# Autodesk Inventor assembly: Gripper2
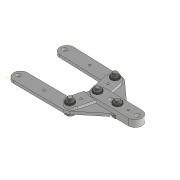
[picture p0: Inventor's stored thumbnail of the model, 180x180]
Saved by Autodesk Inventor 2021 (Build 250183000, 183)
## iProperties
Created: 2022-10-02
Part Number: Gripper2
Document SubType Name: Assembly
Designer: brian
Author: brian
## Documents named in this file (8)
- G:\Mi unidad\Universidad\Control\Robotica\Laboratorio\Proyecto\Gripper2.iam
- G:\Mi unidad\Universidad\Control\Robotica\Laboratorio\Proyecto\GripP1.ipt
- G:\Mi unidad\Universidad\Control\Robotica\Laboratorio\Proyecto\GripP3.ipt
- G:\Mi unidad\Universidad\Control\Robotica\Laboratorio\Proyecto\GripP4.ipt
- C:\Users\brian\OneDrive\Documents\Inventor\Content Center Files\R2021\en-US\ISO 8738(2)\ISO 8738 - 10(2).ipt
- C:\Users\brian\OneDrive\Documents\Inventor\Content Center Files\R2021\en-US\ISO 4017(1)\ISO 4017 - M10 x 20 - ISO.ipt
- C:\Users\brian\OneDrive\Documents\Inventor\Content Center Files\R2021\en-US\ISO 4017(1)\ISO 4017 - M10 x 25 - ISO.ipt
- C:\Users\brian\OneDrive\Documents\Inventor\Content Center Files\R2021\en-US\ISO 8675(2)\ISO 8675 - M8 x 1 - ISO.ipt
## Components (21 placed, 7 different names)
1. GripP1:1 — Rotational:5, Rotational:7, Insert:1, Insert:4
2. GripP3:1 — Rotational:3, Rotational:5, Rotational:6, Insert:10
3. GripP1:2 — Rotational:4, Rotational:7, Tangent:1, Insert:3
4. GripP3:2 — Rotational:3, Rotational:4, Insert:2, Insert:11
5. GripP4:2 — Rotational:6, Tangent:1, Insert:6
6. ISO 8738 10:1 — Insert:1, Insert:9
7. ISO 8738 10:2 — Insert:2, Insert:5
8. ISO 8738 10:3 — Insert:3, Insert:8
9. ISO 8738 10:4 — Insert:4, Insert:7
10. ISO 4017 M10 x 20:1 — Insert:5, Mate:1
11. ISO 8738 10:5 — Insert:6, Mate:2
12. ISO 8675 M8 x 1:1 — Mate:1, Mate:2
13. ISO 4017 M10 x 25:1 — Insert:7
14. ISO 4017 M10 x 25:2 — Insert:8
15. ISO 4017 M10 x 25:3 — Insert:9, Insert:14, Insert:12
16. ISO 8738 10:6 — Insert:10, Insert:15
17. ISO 8738 10:7 — Insert:11, Insert:13
18. ISO 8738 10:8 — Insert:12
19. ISO 8675 M8 x 1:2 — Insert:13
20. ISO 8675 M8 x 1:3 — Insert:14
21. ISO 8675 M8 x 1:4 — Insert:15
## Relationships (23: Insert 15, RevoluteJoint 5, Mate 2, Tangent 1)
- Rotational:3 [RevoluteJoint]: GripP3:1 ↔ GripP3:2
- Rotational:4 [RevoluteJoint]: GripP1:2 ↔ GripP3:2
- Rotational:5 [RevoluteJoint]: GripP1:1 ↔ GripP3:1
- Rotational:6 [RevoluteJoint]: GripP3:1 ↔ GripP4:2
- Rotational:7 [RevoluteJoint]: GripP1:1 ↔ GripP1:2
- Tangent:1: GripP1:2 ↔ GripP4:2
- Insert:1: GripP1:1 ↔ ISO 8738 10:1
- Insert:2: GripP3:2 ↔ ISO 8738 10:2
- Insert:3: GripP1:2 ↔ ISO 8738 10:3
- Insert:4: GripP1:1 ↔ ISO 8738 10:4
- Insert:5: ISO 8738 10:2 ↔ ISO 4017 M10 x 20:1
- Insert:6: GripP4:2 ↔ ISO 8738 10:5
- Mate:1: ISO 4017 M10 x 20:1 ↔ ISO 8675 M8 x 1:1
- Mate:2: ISO 8738 10:5 ↔ ISO 8675 M8 x 1:1
- Insert:7: ISO 8738 10:4 ↔ ISO 4017 M10 x 25:1
- Insert:8: ISO 8738 10:3 ↔ ISO 4017 M10 x 25:2
- Insert:9: ISO 8738 10:1 ↔ ISO 4017 M10 x 25:3
- Insert:10: GripP3:1 ↔ ISO 8738 10:6
- Insert:11: GripP3:2 ↔ ISO 8738 10:7
- Insert:12 (-5 mm): ISO 4017 M10 x 25:3 ↔ ISO 8738 10:8
- Insert:13: ISO 8738 10:7 ↔ ISO 8675 M8 x 1:2
- Insert:14 (-5 mm): ISO 4017 M10 x 25:3 ↔ ISO 8675 M8 x 1:3
- Insert:15: ISO 8738 10:6 ↔ ISO 8675 M8 x 1:4
